# Autodesk Inventor assembly: chest_cover
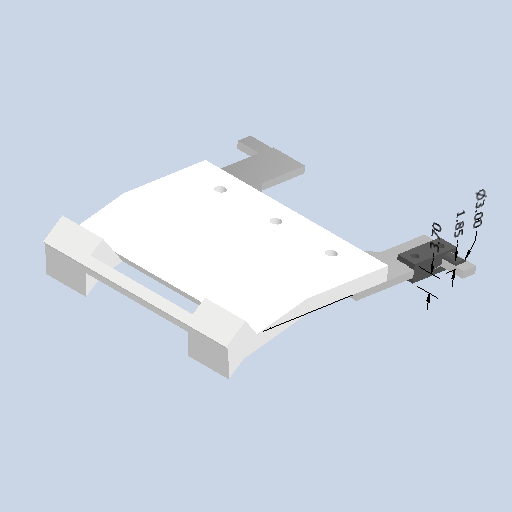
[picture p0: Inventor's stored thumbnail of the model, 512x512]
Saved by Autodesk Inventor 2026.1 (Build 301233020, 233B)
## iProperties
Created: 2024-10-12
Part Number: chest_cover
Document SubType Name: Assembly
Designer: hibik
Author: hibik
## Documents named in this file (4)
- C:\Users\hibik\Documents\Robomech\HR\Eglantyne_mark2\hard\upper_body\chest\chest_cover.iam
- C:\Users\hibik\Documents\Robomech\HR\Eglantyne_mark2\hard\upper_body\chest\chest_cover_base.ipt
- C:\Users\hibik\Documents\Robomech\HR\Eglantyne_mark2\hard\upper_body\chest\chest_cover_axis_right.ipt
- C:\Users\hibik\Documents\Robomech\HR\Eglantyne_mark2\hard\upper_body\chest\chest_cover_front.ipt
## Components (3 placed, 3 different names)
1. chest_cover_base:1 — メイト:1, フラッシュ:1, フラッシュ:2, 挿入:1, 角度:1
2. chest_cover_axis_right:1 — メイト:1, フラッシュ:1, フラッシュ:2
3. chest_cover_front:1 — 挿入:1, 角度:1
## Relationships (5: Flush 2, Mate 1, Insert 1, Angle 1)
- メイト:1 [Mate] (0.1 mm): chest_cover_base:1 ↔ chest_cover_axis_right:1
- フラッシュ:1 [Flush]: chest_cover_base:1 ↔ chest_cover_axis_right:1
- フラッシュ:2 [Flush]: chest_cover_base:1 ↔ chest_cover_axis_right:1
- 挿入:1 [Insert]: chest_cover_base:1 ↔ chest_cover_front:1
- 角度:1 [Angle] (180 deg): chest_cover_base:1 ↔ chest_cover_front:1
